# Autodesk Inventor assembly: gusset_mirrored
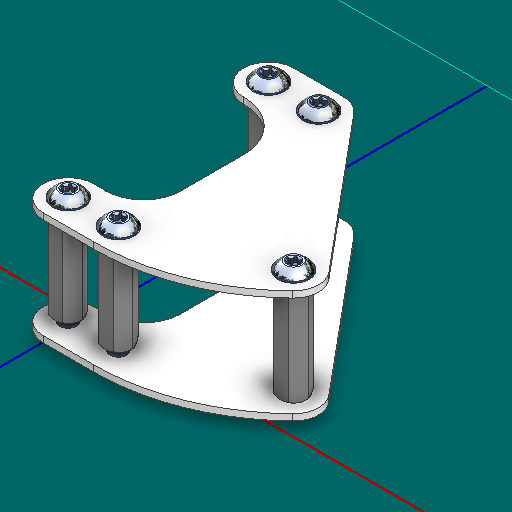
[picture p0: Inventor's stored thumbnail of the model, 512x512]
Saved by Autodesk Inventor 2025 (Build 290162000, 162)
## iProperties
Created: 2024-08-21
Part Number: gusset_mirrored
Document SubType Name: Assembly
Designer: averey
Author: averey
## Documents named in this file (9)
- C:\Users\avere\vex_robotics_high_stakes\hardware\cad\bots\ENIGMA\chassis\drivetrain\drivebay_mirrored\gusset_mirrored.iam
- C:\Users\avere\vex_robotics_high_stakes\hardware\cad\bots\ENIGMA\chassis\drivetrain\drivebay_mirrored\gusset_mirrored.ipt
- C:\Users\avere\vex_robotics_high_stakes\hardware\cad\VEX-CAD-Inventor\Structure\Standoff\Standoff 1.00.ipt
- C:\Users\avere\vex_robotics_high_stakes\hardware\cad\VEX-CAD-Inventor\Structure\Standoff.ipt
- C:\Users\avere\vex_robotics_high_stakes\hardware\cad\VEX-CAD-Inventor\Structure\Standoff\Standoff .875.ipt
- C:\Users\avere\vex_robotics_high_stakes\hardware\cad\VEX-CAD-Inventor\Structure\Hardware\Screw Shoulder Robosource\SScrew Shoulder Smooth .290 x .09.ipt
- C:\Users\avere\vex_robotics_high_stakes\hardware\cad\VEX-CAD-Inventor\Structure\Hardware\Screw Shoulder Robosource.ipt
- C:\Users\avere\vex_robotics_high_stakes\hardware\cad\VEX-CAD-Inventor\Structure\Hardware\Screw Steel - Star\SScrew Star Smooth .250.ipt
- C:\Users\avere\vex_robotics_high_stakes\hardware\cad\VEX-CAD-Inventor\Structure\Hardware\Screw Steel - Star.ipt
## Components (17 placed, 5 different names)
1. gusset_mirrored:1 — Mate:1, Insert:1, Insert:3, Insert:4, Insert:6
2. gusset_mirrored:2 — Mate:1, Insert:1, Insert:2, Insert:5, Insert:7
3. Standoff 1.00:1 — Insert:2
4. SScrew Star Smooth .250:1 — Insert:7
5. SScrew Star Smooth .250:2 — Insert:6
6. Standoff .875:2 — Insert:3
7. Standoff .875:3
8. Standoff .875:4
9. Standoff .875:5
10. SScrew Shoulder Smooth .290 x .09:1 — Insert:4
11. SScrew Shoulder Smooth .290 x .09:3
12. SScrew Shoulder Smooth .290 x .09:4
13. SScrew Shoulder Smooth .290 x .09:5
14. SScrew Shoulder Smooth .290 x .09:2 — Insert:5
15. SScrew Shoulder Smooth .290 x .09:6
16. SScrew Shoulder Smooth .290 x .09:7
17. SScrew Shoulder Smooth .290 x .09:8
## Component patterns: (4 elements, first: Standoff .875:2), (4 elements, first: SScrew Shoulder Smooth .290 x .09:1), (4 elements, first: SScrew Shoulder Smooth .290 x .09:2)
## Relationships (8: Insert 7, Mate 1)
- Mate:1: gusset_mirrored:1 ↔ gusset_mirrored:2
- Insert:1 (25.4 mm): gusset_mirrored:1 ↔ gusset_mirrored:2
- Insert:2: gusset_mirrored:2 ↔ Standoff 1.00:1
- Insert:3 (1.5875 mm): gusset_mirrored:1 ↔ Standoff .875:2
- Insert:4: gusset_mirrored:1 ↔ SScrew Shoulder Smooth .290 x .09:1
- Insert:5: gusset_mirrored:2 ↔ SScrew Shoulder Smooth .290 x .09:2
- Insert:7: gusset_mirrored:2 ↔ SScrew Star Smooth .250:1
- Insert:6: gusset_mirrored:1 ↔ SScrew Star Smooth .250:2
